# Autodesk Inventor assembly: Electronic Assembly
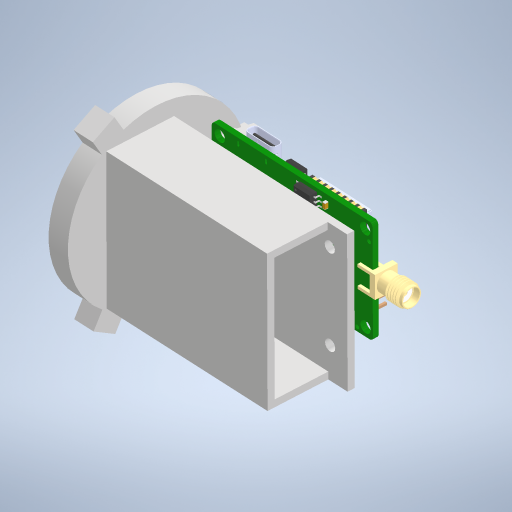
[picture p0: Inventor's stored thumbnail of the model, 512x512]
Saved by Autodesk Inventor 2024 (Build 280153000, 153)
## iProperties
Created: 2024-04-22
Part Number: Electronic Assembly
Document SubType Name: Assembly
Designer: auror
Author: auror
## Documents named in this file (3)
- C:\Users\auror\Documents\TU Delft\DARE\Git\Scrambler-2-CAD\Autodesk\Electronic Assembly.iam
- C:\Users\auror\Documents\TU Delft\DARE\Git\Scrambler-2-CAD\Autodesk\Electronic casing.ipt
- C:\Users\auror\Documents\TU Delft\DARE\Git\Scrambler-2-CAD\Autodesk\Kolibri\Kolibri_rev1.1.iam
## Components (2 placed, 2 different names)
1. Electronic casing:1 — Mate:1, Mate:2, Mate:3, Mate:4, Mate:5
2. Kolibri_rev1.1:1 [sub-assembly] — Mate:1, Mate:2, Mate:3, Mate:4, Mate:5
## Relationships (5: Mate 5)
- Mate:1: Electronic casing:1 ↔ Kolibri_rev1.1:1
- Mate:2: Electronic casing:1 ↔ Kolibri_rev1.1:1
- Mate:3: Electronic casing:1 ↔ Kolibri_rev1.1:1
- Mate:4: Electronic casing:1 ↔ Kolibri_rev1.1:1
- Mate:5: Electronic casing:1 ↔ Kolibri_rev1.1:1
